# Autodesk Inventor assembly: enclosure_asus.ipt
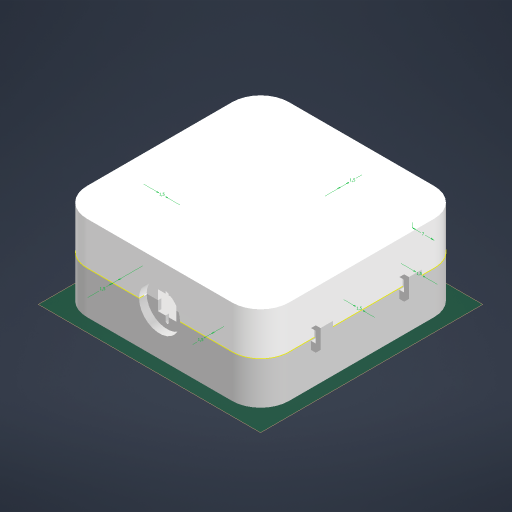
[picture p0: Inventor's stored thumbnail of the model, 512x512]
Saved by Autodesk Inventor 2024.1 (Build 281209000, 209)
## iProperties
Created: 2023-07-19
Part Number: enclosure_asus.ipt
Document SubType Name: Assembly
Designer: LabTel_Admin
Author: LabTel_Admin
## Documents named in this file (3)
- C:\Users\LabTel_Admin\Documents\Inventor\Projects\enclosure_asus\enclosure_asus_asembly.ipt.iam
- C:\Users\LabTel_Admin\Documents\Inventor\Projects\enclosure_asus\enclosure_down.ipt
- C:\Users\LabTel_Admin\Documents\Inventor\Projects\enclosure_asus\enclosure_up.ipt
## Components (2 placed, 2 different names)
1. enclosure_down:1 — Mate:2, Flush:3, Flush:4
2. enclosure_up:1 — Mate:2, Flush:3, Flush:4
## Relationships (3: Flush 2, Mate 1)
- Mate:2: enclosure_down:1 ↔ enclosure_up:1
- Flush:3: enclosure_down:1 ↔ enclosure_up:1
- Flush:4: enclosure_down:1 ↔ enclosure_up:1
